# Autodesk Inventor assembly: reductor_10_6_ass
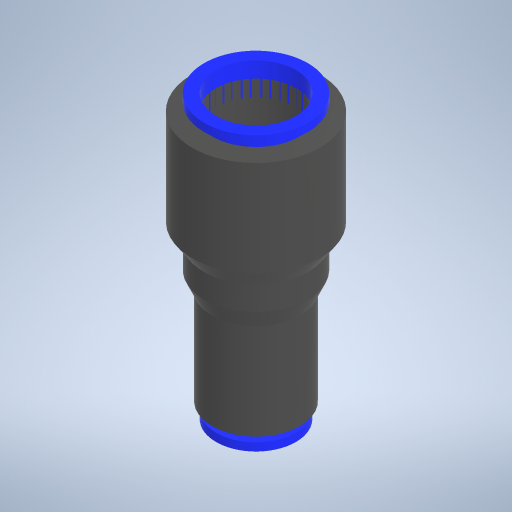
[picture p0: Inventor's stored thumbnail of the model, 512x512]
Saved by Autodesk Inventor 2024 (Build 280153000, 153)
## iProperties
Created: 2023-04-11
Part Number: reductor_10_6_ass
Document SubType Name: Assembly
Designer: ferna
Author: ferna
## Documents named in this file (4)
- C:\Users\ferna\OneDrive - Universidad Católica de Chile\Bocas\RobotFlautista\reductor_10_6_ass.iam
- C:\Users\ferna\OneDrive - Universidad Católica de Chile\Bocas\RobotFlautista\entrada_manguera_6.ipt
- C:\Users\ferna\OneDrive - Universidad Católica de Chile\Bocas\RobotFlautista\reductor_10_6.ipt
- C:\Users\ferna\OneDrive - Universidad Católica de Chile\Bocas\RobotFlautista\entrada_manguera_2.ipt
## Components (3 placed, 3 different names)
1. entrada_manguera_6:1 — Mate:1, Mate:2
2. reductor_10_6:1 — Mate:1, Mate:2, Mate:3, Mate:4
3. entrada_manguera_2:1 — Mate:3, Mate:4
## Relationships (4: Mate 4)
- Mate:1 (-2.032 mm): entrada_manguera_6:1 ↔ reductor_10_6:1
- Mate:2: entrada_manguera_6:1 ↔ reductor_10_6:1
- Mate:3 (-2.032 mm): reductor_10_6:1 ↔ entrada_manguera_2:1
- Mate:4: reductor_10_6:1 ↔ entrada_manguera_2:1
